# Autodesk Inventor assembly: V-GROVE,TEST
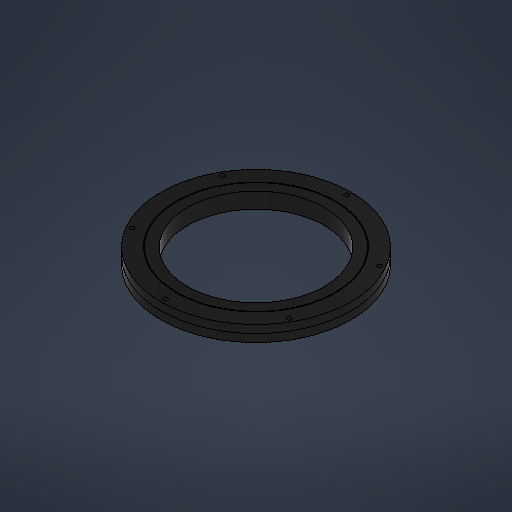
[picture p0: Inventor's stored thumbnail of the model, 512x512]
Saved by Autodesk Inventor 2026 (Build 300175000, 175)
## iProperties
Created: 2026-02-03
Part Number: V-GROVE,TEST
Document SubType Name: Assembly
Designer: littl
Author: littl
## Documents named in this file (4)
- C:\Users\littl\OneDrive\Documents\GitHub\2026-Robot-Mechanical\Shooter\Turret\V-GROVE,TEST.iam
- C:\Users\littl\OneDrive\Documents\GitHub\2026-Robot-Mechanical\Shooter\Turret\3DPRINT,OUTER-V.ipt
- C:\Users\littl\OneDrive\Documents\GitHub\2026-Robot-Mechanical\Shooter\Turret\3DPRINT,INNER-V.ipt
- C:\Users\littl\OneDrive\Documents\GitHub\2026-Robot-Mechanical\#1_CAD Library\Miscellaneous\PURCHASED,7.237ID,0.103inWIDTH,O-RING.ipt
## Components (5 placed, 3 different names)
1. 3DPRINT,OUTER-V:1 — Mate:1, Flush:1, Mate:2, Mate:3, Mate:4, Mate:6, Mate:7, Mate:8, Mate:10
2. 3DPRINT,INNER-V:1 — Mate:1, Flush:1, Mate:8
3. PURCHASED,7.237ID,0.103inWIDTH,O-RING:1 — Mate:2
4. PURCHASED,7.237ID,0.103inWIDTH,O-RING:2 — Mate:3
5. 3DPRINT,OUTER-V:2 — Mate:6, Mate:7, Mate:9, Mate:10
## Relationships (10: Mate 9, Flush 1)
- Mate:1: 3DPRINT,OUTER-V:1 ↔ 3DPRINT,INNER-V:1
- Flush:1: 3DPRINT,OUTER-V:1 ↔ 3DPRINT,INNER-V:1
- Mate:2: 3DPRINT,OUTER-V:1 ↔ PURCHASED,7.237ID,0.103inWIDTH,O-RING:1
- Mate:3: 3DPRINT,OUTER-V:1 ↔ PURCHASED,7.237ID,0.103inWIDTH,O-RING:2
- Mate:4: 3DPRINT,OUTER-V:1
- Mate:6: 3DPRINT,OUTER-V:1 ↔ 3DPRINT,OUTER-V:2
- Mate:7: 3DPRINT,OUTER-V:1 ↔ 3DPRINT,OUTER-V:2
- Mate:8: 3DPRINT,OUTER-V:1 ↔ 3DPRINT,INNER-V:1
- Mate:9: 3DPRINT,OUTER-V:2
- Mate:10: 3DPRINT,OUTER-V:1 ↔ 3DPRINT,OUTER-V:2
